# Autodesk Inventor assembly: Forward Shell
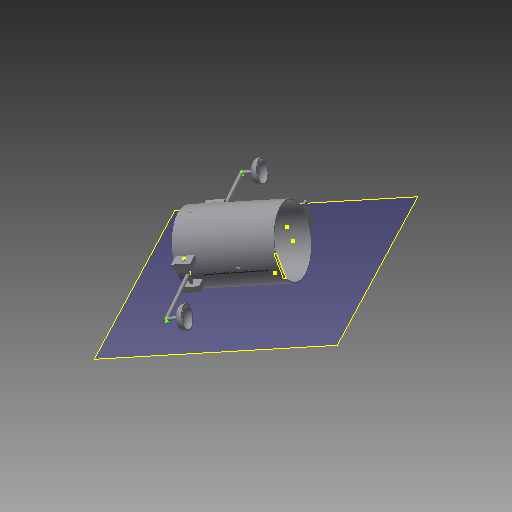
[picture p0: Inventor's stored thumbnail of the model, 512x512]
Saved by Autodesk Inventor 2018 (Build 220112000, 112)
## iProperties
Created: 2021-03-15
Part Number: Forward Shell
Document SubType Name: Assembly
Designer: vishal
Author: vishal
## Documents named in this file (4)
- C:\Users\dell\Desktop\ES101 GROUP-13 PROJECT\FINAL MODEL\Resolved files\Forward Shell.iam
- C:\Users\dell\Desktop\ES101 GROUP-13 PROJECT\INDIVIDUAL WORK\Vishal\Resolved Parts\forward shell Part1.ipt
- C:\Users\dell\Desktop\ES101 GROUP-13 PROJECT\INDIVIDUAL WORK\Vishal\Resolved Parts\Forward Shell part 2.ipt
- C:\Users\dell\Desktop\ES101 GROUP-13 PROJECT\INDIVIDUAL WORK\Dhruv\magnetic torquer.ipt
## Components (5 placed, 3 different names)
1. forward shell Part1:1 — Mate:1, Mate:2, Mate:3, Mate:4, Flush:1, Mate:6, Mate:7, Mate:8, Mate:9, Mate:10, Mate:11, Mate:12
2. Forward Shell part 2:1 — Mate:3, Mate:4
3. Forward Shell part 2:2 — Mate:1, Mate:2
4. magnetic torquer:2 — Mate:6, Mate:7, Mate:8
5. magnetic torquer:3 — Mate:9, Mate:10, Mate:11, Mate:12
## Relationships (12: Mate 11, Flush 1)
- Mate:1: forward shell Part1:1 ↔ Forward Shell part 2:2
- Mate:2: forward shell Part1:1 ↔ Forward Shell part 2:2
- Mate:3: forward shell Part1:1 ↔ Forward Shell part 2:1
- Mate:4: forward shell Part1:1 ↔ Forward Shell part 2:1
- Flush:1 (88.9 mm): forward shell Part1:1
- Mate:6: forward shell Part1:1 ↔ magnetic torquer:2
- Mate:7: forward shell Part1:1 ↔ magnetic torquer:2
- Mate:8 (27.5082 mm): forward shell Part1:1 ↔ magnetic torquer:2
- Mate:9: forward shell Part1:1 ↔ magnetic torquer:3
- Mate:10: forward shell Part1:1 ↔ magnetic torquer:3
- Mate:11 (27.5082 mm): forward shell Part1:1 ↔ magnetic torquer:3
- Mate:12 (27.5082 mm): forward shell Part1:1 ↔ magnetic torquer:3
